# Autodesk Inventor assembly: Chassis Assembly
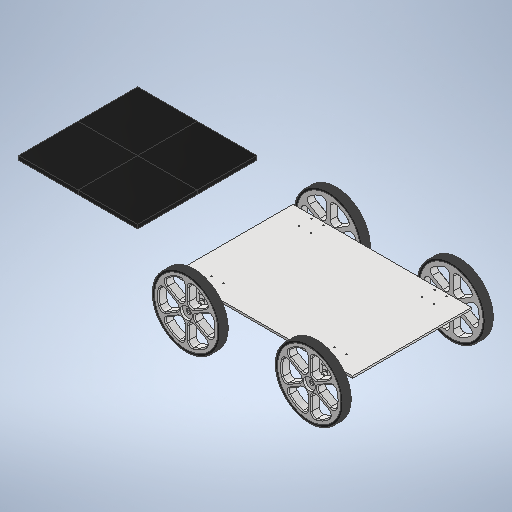
[picture p0: Inventor's stored thumbnail of the model, 512x512]
Saved by Autodesk Inventor 2025.2 (Build 292293000, 293)
## iProperties
Created: 2025-01-16
Part Number: Chassis Assembly
Document SubType Name: Assembly
Designer: Matt Tidd
Author: Matt Tidd
## Documents named in this file (8)
- C:\Users\mtidd\OneDrive\Desktop\H2A\CAD\Chassis_Design\Chassis Assembly.iam
- C:\Users\mtidd\OneDrive\Desktop\H2A\CAD\Motors_and_Wheels\520 DC Gear Motor Bracket Assembly.iam
- C:\Users\mtidd\OneDrive\Desktop\H2A\CAD\Chassis_Design\ChassisTest.ipt
- C:\Users\mtidd\OneDrive\Desktop\H2A\CAD\Motors_and_Wheels\520 DC Gear Motor Wheel Coupler.ipt
- C:\Users\mtidd\OneDrive\Desktop\H2A\CAD\Motors_and_Wheels\PLA Wheel Frame.ipt
- C:\Users\mtidd\OneDrive\Desktop\H2A\CAD\Motors_and_Wheels\TPU Tire.ipt
- C:\Users\mtidd\OneDrive\Desktop\H2A\CAD\TrashStorageUnit\TSU - V2\TSU_FM_Floor.ipt
- C:\Users\mtidd\OneDrive\Desktop\H2A\CAD\TrashStorageUnit\TSU - V2\TSU_MF_Floor.ipt
## Components (21 placed, 7 different names)
1. ChassisTest:1 — Mate:1, Mate:2, Mate:3, Mate:4, Mate:5, Mate:6, Mate:7, Mate:8
2. 520 DC Gear Motor Bracket Assembly:1 [sub-assembly] — Mate:1, Mate:2, Mate:10
3. 520 DC Gear Motor Bracket Assembly:2 [sub-assembly] — Mate:3, Mate:4, Mate:9
4. 520 DC Gear Motor Bracket Assembly:3 [sub-assembly] — Mate:7, Mate:8, Mate:11
5. 520 DC Gear Motor Bracket Assembly:4 [sub-assembly] — Mate:5, Mate:6, Mate:12
6. 520 DC Gear Motor Wheel Coupler:1 — Mate:9, Mate:17, Mate:18
7. 520 DC Gear Motor Wheel Coupler:2 — Mate:10, Mate:19, Mate:20
8. 520 DC Gear Motor Wheel Coupler:3 — Mate:11, Mate:15, Mate:16
9. 520 DC Gear Motor Wheel Coupler:4 — Mate:12, Mate:13, Mate:14
10. PLA Wheel Frame:1 — Mate:15, Mate:16, Mate:24
11. PLA Wheel Frame:2 — Mate:13, Mate:14, Mate:23
12. PLA Wheel Frame:3 — Mate:19, Mate:20, Mate:21
13. PLA Wheel Frame:4 — Mate:17, Mate:18, Mate:22
14. TPU Tire:1 — Mate:21
15. TPU Tire:2 — Mate:24
16. TPU Tire:3 — Mate:23
17. TPU Tire:4 — Mate:22
18. TSU_FM_Floor:1 — Mate:27, Mate:28, Mate:29, Mate:30
19. TSU_MF_Floor:1 — Mate:27, Mate:28
20. TSU_FM_Floor:2 — Mate:25, Mate:26, Mate:29, Mate:30
21. TSU_MF_Floor:2 — Mate:25, Mate:26
## Relationships (30: Mate 30)
- Mate:1: ChassisTest:1 ↔ 520 DC Gear Motor Bracket Assembly:1
- Mate:2 (50 mm): ChassisTest:1 ↔ 520 DC Gear Motor Bracket Assembly:1
- Mate:3: ChassisTest:1 ↔ 520 DC Gear Motor Bracket Assembly:2
- Mate:4 (50 mm): ChassisTest:1 ↔ 520 DC Gear Motor Bracket Assembly:2
- Mate:5 (50 mm): ChassisTest:1 ↔ 520 DC Gear Motor Bracket Assembly:4
- Mate:6: ChassisTest:1 ↔ 520 DC Gear Motor Bracket Assembly:4
- Mate:7: ChassisTest:1 ↔ 520 DC Gear Motor Bracket Assembly:3
- Mate:8 (50 mm): ChassisTest:1 ↔ 520 DC Gear Motor Bracket Assembly:3
- Mate:9: 520 DC Gear Motor Bracket Assembly:2 ↔ 520 DC Gear Motor Wheel Coupler:1
- Mate:10: 520 DC Gear Motor Bracket Assembly:1 ↔ 520 DC Gear Motor Wheel Coupler:2
- Mate:11: 520 DC Gear Motor Bracket Assembly:3 ↔ 520 DC Gear Motor Wheel Coupler:3
- Mate:12: 520 DC Gear Motor Bracket Assembly:4 ↔ 520 DC Gear Motor Wheel Coupler:4
- Mate:13: 520 DC Gear Motor Wheel Coupler:4 ↔ PLA Wheel Frame:2
- Mate:14: 520 DC Gear Motor Wheel Coupler:4 ↔ PLA Wheel Frame:2
- Mate:15: 520 DC Gear Motor Wheel Coupler:3 ↔ PLA Wheel Frame:1
- Mate:16: 520 DC Gear Motor Wheel Coupler:3 ↔ PLA Wheel Frame:1
- Mate:17: 520 DC Gear Motor Wheel Coupler:1 ↔ PLA Wheel Frame:4
- Mate:18: 520 DC Gear Motor Wheel Coupler:1 ↔ PLA Wheel Frame:4
- Mate:19: 520 DC Gear Motor Wheel Coupler:2 ↔ PLA Wheel Frame:3
- Mate:20: 520 DC Gear Motor Wheel Coupler:2 ↔ PLA Wheel Frame:3
- Mate:21: PLA Wheel Frame:3 ↔ TPU Tire:1
- Mate:22: PLA Wheel Frame:4 ↔ TPU Tire:4
- Mate:23: PLA Wheel Frame:2 ↔ TPU Tire:3
- Mate:24: PLA Wheel Frame:1 ↔ TPU Tire:2
- Mate:25: TSU_FM_Floor:2 ↔ TSU_MF_Floor:2
- Mate:26: TSU_FM_Floor:2 ↔ TSU_MF_Floor:2
- Mate:27: TSU_FM_Floor:1 ↔ TSU_MF_Floor:1
- Mate:28: TSU_FM_Floor:1 ↔ TSU_MF_Floor:1
- Mate:29: TSU_FM_Floor:1 ↔ TSU_FM_Floor:2
- Mate:30: TSU_FM_Floor:1 ↔ TSU_FM_Floor:2
